# Autodesk Inventor assembly: Ensemble1
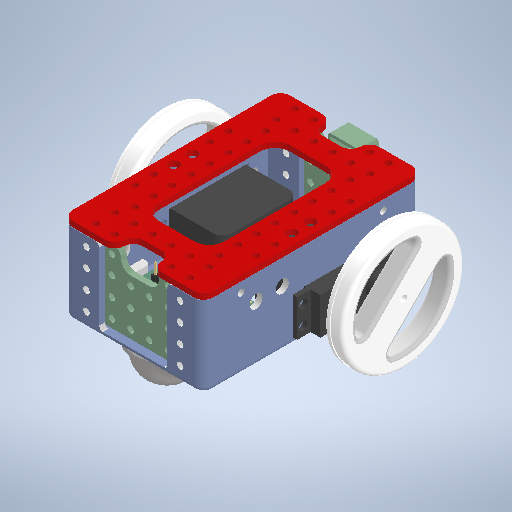
[picture p0: Inventor's stored thumbnail of the model, 512x512]
Saved by Autodesk Inventor 2025 (Build 290162000, 162)
## iProperties
Created: 2024-09-06
Part Number: Ensemble1
Document SubType Name: Assembly
Designer: chass
Author: chass
## Documents named in this file (10)
- C:\Users\chass\Documents\AREM\Hackathon_2024\Modeles_3D\Ensemble1.iam
- C:\Users\chass\Documents\AREM\Hackathon_2024\Modeles_3D\chassis.ipt
- C:\Users\chass\Documents\AREM\Hackathon_2024\Modeles_3D\servomoteur_roues.ipt
- C:\Users\chass\Documents\AREM\Hackathon_2024\Modeles_3D\plaque.ipt
- C:\Users\chass\Documents\AREM\Hackathon_2024\Modeles_3D\roue.ipt
- C:\Users\chass\Documents\AREM\Hackathon_2024\Modeles_3D\support_tof_actionneur_panneaux_solaires.ipt
- C:\Users\chass\Documents\AREM\Hackathon_2024\Modeles_3D\roulette.ipt
- C:\Users\chass\Documents\AREM\Hackathon_2024\Modeles_3D\toit.ipt
- C:\Users\chass\Documents\AREM\Hackathon_2024\PCB\pcb_robot\pcb_robot\pcb_robot_v2.iam
- C:\Users\chass\Documents\AREM\Hackathon_2024\Modeles_3D\pare-chocs.ipt
## Components (12 placed, 9 different names)
1. chassis:1 — Placage:1, Placage:2, Placage:3, Placage:4, Placage:5, Placage:6, Placage:7, Placage:8, Placage:9, Placage:10, Placage:11, Placage:12, Placage:22, Placage:23, Placage:24, Placage:25, Placage:26, Placage:28, Placage:29, Placage:30, Placage:31, Placage:32, Placage:33
2. servomoteur_roues:1 — Placage:4, Placage:5, Placage:6, Placage:15
3. servomoteur_roues:2 — Placage:1, Placage:2, Placage:3, Placage:13, Placage:14
4. plaque:1 — Placage:7, Placage:8, Placage:9, Placage:18, Placage:19, Placage:20
5. plaque:2 — Placage:10, Placage:11, Placage:12
6. roue:1 — Placage:13, Placage:14
7. roue:2 — Placage:15
8. support_tof_actionneur_panneaux_solaires:1 — Placage:18, Placage:19, Placage:20
9. roulette:1 — Placage:22, Placage:23
10. toit:1 — Placage:24, Placage:25, Placage:26
11. pcb_robot_v2:1 [sub-assembly] — Placage:28, Placage:29, Placage:30
12. pare-chocs:1 — Placage:31, Placage:32, Placage:33
## Relationships (29: Mate 29)
- Placage:1 [Mate]: chassis:1 ↔ servomoteur_roues:2
- Placage:2 [Mate]: chassis:1 ↔ servomoteur_roues:2
- Placage:3 [Mate]: chassis:1 ↔ servomoteur_roues:2
- Placage:4 [Mate]: chassis:1 ↔ servomoteur_roues:1
- Placage:5 [Mate]: chassis:1 ↔ servomoteur_roues:1
- Placage:6 [Mate]: chassis:1 ↔ servomoteur_roues:1
- Placage:7 [Mate]: chassis:1 ↔ plaque:1
- Placage:8 [Mate]: chassis:1 ↔ plaque:1
- Placage:9 [Mate]: chassis:1 ↔ plaque:1
- Placage:10 [Mate]: chassis:1 ↔ plaque:2
- Placage:11 [Mate]: chassis:1 ↔ plaque:2
- Placage:12 [Mate]: chassis:1 ↔ plaque:2
- Placage:13 [Mate]: servomoteur_roues:2 ↔ roue:1
- Placage:14 [Mate]: servomoteur_roues:2 ↔ roue:1
- Placage:15 [Mate]: servomoteur_roues:1 ↔ roue:2
- Placage:18 [Mate]: plaque:1 ↔ support_tof_actionneur_panneaux_solaires:1
- Placage:19 [Mate]: plaque:1 ↔ support_tof_actionneur_panneaux_solaires:1
- Placage:20 [Mate]: plaque:1 ↔ support_tof_actionneur_panneaux_solaires:1
- Placage:22 [Mate]: chassis:1 ↔ roulette:1
- Placage:23 [Mate]: chassis:1 ↔ roulette:1
- Placage:24 [Mate]: chassis:1 ↔ toit:1
- Placage:25 [Mate]: chassis:1 ↔ toit:1
- Placage:26 [Mate]: chassis:1 ↔ toit:1
- Placage:28 [Mate]: chassis:1 ↔ pcb_robot_v2:1
- Placage:29 [Mate]: chassis:1 ↔ pcb_robot_v2:1
- Placage:30 [Mate]: chassis:1 ↔ pcb_robot_v2:1
- Placage:31 [Mate]: chassis:1 ↔ pare-chocs:1
- Placage:32 [Mate]: chassis:1 ↔ pare-chocs:1
- Placage:33 [Mate]: chassis:1 ↔ pare-chocs:1
